# Autodesk Inventor assembly: Bearing
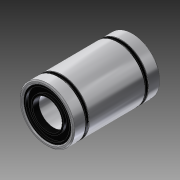
[picture p0: Inventor's stored thumbnail of the model, 180x180]
Saved by Autodesk Inventor 2014 SP1 (Build 180222100, 222)
## iProperties
Created: 2017-07-23
Part Number: Bearing
Document SubType Name: Assembly
Designer: Stepan
Author: Stepan
## Documents named in this file (4)
- D:\3DPrinter\LMUU\Bearing.iam
- D:\3DPrinter\LMUU\bearing.ipt
- D:\3DPrinter\LMUU\rubber.ipt
- D:\3DPrinter\LMUU\Cap.ipt
## Components (5 placed, 3 different names)
1. bearing:1 — Совмещение:1, Совмещение:2, Совмещение:3, Совмещение:4, Заподлицо:1, Совмещение:5, Совмещение:6, Совмещение:8
2. rubber:1 — Совмещение:3, Совмещение:4
3. rubber:2 — Совмещение:1, Совмещение:2
4. Cap:1 — Заподлицо:1, Совмещение:5
5. Cap:2 — Совмещение:6, Совмещение:8
## Relationships (8: Mate 7, Flush 1)
- Совмещение:1 [Mate]: bearing:1 ↔ rubber:2
- Совмещение:2 [Mate]: bearing:1 ↔ rubber:2
- Совмещение:3 [Mate]: bearing:1 ↔ rubber:1
- Совмещение:4 [Mate]: bearing:1 ↔ rubber:1
- Заподлицо:1 [Flush]: bearing:1 ↔ Cap:1
- Совмещение:5 [Mate]: bearing:1 ↔ Cap:1
- Совмещение:6 [Mate]: bearing:1 ↔ Cap:2
- Совмещение:8 [Mate]: bearing:1 ↔ Cap:2
